# Autodesk Inventor assembly: Eje Final
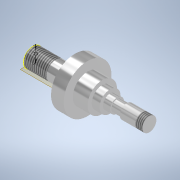
[picture p0: Inventor's stored thumbnail of the model, 180x180]
Saved by Autodesk Inventor 2021 (Build 250183000, 183)
## iProperties
Created: 2021-01-01
Part Number: Eje Final
Document SubType Name: Assembly
Designer: dieku
Author: dieku
## Documents named in this file (5)
- C:\Users\dieku\Documents\GitHub\tallerDibujoIngenieria\Partes\Eje\Eje Final.iam
- C:\Users\dieku\Documents\GitHub\tallerDibujoIngenieria\Partes\Eje\Intento 1-1-2021\5 Cilindros centrales.ipt
- C:\Users\dieku\Documents\GitHub\tallerDibujoIngenieria\Partes\Eje\Intento 1-1-2021\Cilindro Final diametro 20 largo 32.ipt
- C:\Users\dieku\Documents\GitHub\tallerDibujoIngenieria\Partes\Eje\Intento 1-1-2021\Cilindro Inicial con Corte.ipt
- C:\Users\dieku\Documents\GitHub\tallerDibujoIngenieria\Partes\CHAVETA UNE 17012 8X7X20.ipt
## Components (4 placed, 4 different names)
1. 5 Cilindros centrales:1 — Insert:1, Insert:2
2. Cilindro Final diametro 20 largo 32:1 — Insert:1
3. Cilindro Inicial con Corte:1 — Insert:2, Mate:1, Mate:2, Mate:3
4. CHAVETA UNE 17012 8X7X20:1 — Mate:1, Mate:2, Mate:3
## Relationships (5: Mate 3, Insert 2)
- Insert:1: 5 Cilindros centrales:1 ↔ Cilindro Final diametro 20 largo 32:1
- Insert:2: 5 Cilindros centrales:1 ↔ Cilindro Inicial con Corte:1
- Mate:1: Cilindro Inicial con Corte:1 ↔ CHAVETA UNE 17012 8X7X20:1
- Mate:2: Cilindro Inicial con Corte:1 ↔ CHAVETA UNE 17012 8X7X20:1
- Mate:3: Cilindro Inicial con Corte:1 ↔ CHAVETA UNE 17012 8X7X20:1
